# Autodesk Inventor assembly: CE-9.1.1
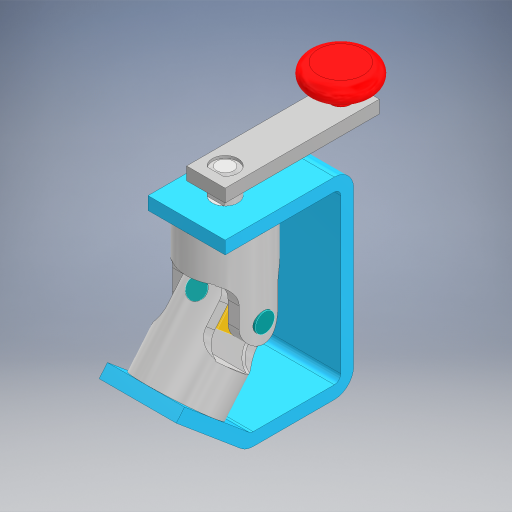
[picture p0: Inventor's stored thumbnail of the model, 512x512]
Saved by Autodesk Inventor 2024 (Build 280153000, 153)
## iProperties
Created: 2024-03-14
Part Number: CE-9.1.1
Document SubType Name: Assembly
Designer: Alex
Author: Alex
## Documents named in this file (9)
- C:\Shared\alex-bartella-schoolwork\4z03\Week 9\CE-9.1.1.iam
- C:\Shared\alex-bartella-schoolwork\4z03\Week 9\STEP\CE-9.1.1 STEP Files\bracket\bracket.ipt
- C:\Shared\alex-bartella-schoolwork\4z03\Week 9\STEP\CE-9.1.1 STEP Files\Yoke_F\Yoke_F.ipt
- C:\Shared\alex-bartella-schoolwork\4z03\Week 9\STEP\CE-9.1.1 STEP Files\Yoke_M\Yoke_M.ipt
- C:\Shared\alex-bartella-schoolwork\4z03\Week 9\STEP\CE-9.1.1 STEP Files\spider\spider.ipt
- C:\Shared\alex-bartella-schoolwork\4z03\Week 9\STEP\CE-9.1.1 STEP Files\arm\arm.ipt
- C:\Shared\alex-bartella-schoolwork\4z03\Week 9\STEP\CE-9.1.1 STEP Files\knob\knob.ipt
- C:\Shared\alex-bartella-schoolwork\4z03\Week 9\STEP\CE-9.1.1 STEP Files\pin_long\pin_long.ipt
- C:\Shared\alex-bartella-schoolwork\4z03\Week 9\STEP\CE-9.1.1 STEP Files\pin_short\pin_short.ipt
## Components (9 placed, 8 different names)
1. bracket:1 — Flush:1, Flush:2, Flush:3, Mate:1, Mate:2, Angle:1, Angle:4
2. Yoke_F:1 — Angle:1, Mate:4, Mate:6, Mate:13
3. Yoke_M:1 — Mate:1, Mate:2, Mate:3, Mate:5, Angle:3, Mate:8, Mate:11, Mate:12, Flush:7
4. spider:1 — Mate:3, Mate:4, Mate:5, Mate:6, Flush:4, Flush:5, Flush:6
5. arm:1 — Angle:3, Mate:8, Mate:9, Mate:10, Flush:7, Angle:4
6. knob:1 — Mate:9, Mate:10
7. pin_long:1 — Mate:13, Flush:6
8. pin_short:1 — Mate:12, Flush:4
9. pin_short:2 — Mate:11, Flush:5
## Relationships (22: Mate 12, Flush 7, Angle 3)
- Flush:1: bracket:1
- Flush:2: bracket:1
- Flush:3: bracket:1
- Mate:1: bracket:1 ↔ Yoke_M:1
- Mate:2: bracket:1 ↔ Yoke_M:1
- Angle:1 (180 deg): bracket:1 ↔ Yoke_F:1
- Mate:3: Yoke_M:1 ↔ spider:1
- Mate:4: Yoke_F:1 ↔ spider:1
- Mate:5 (0.5 mm): Yoke_M:1 ↔ spider:1
- Mate:6 (0.5 mm): Yoke_F:1 ↔ spider:1
- Angle:3 (180 deg): Yoke_M:1 ↔ arm:1
- Mate:8: Yoke_M:1 ↔ arm:1
- Mate:9: arm:1 ↔ knob:1
- Mate:10: arm:1 ↔ knob:1
- Mate:11: Yoke_M:1 ↔ pin_short:2
- Mate:12: Yoke_M:1 ↔ pin_short:1
- Flush:4 (-10 mm): spider:1 ↔ pin_short:1
- Flush:5 (-10 mm): spider:1 ↔ pin_short:2
- Mate:13: Yoke_F:1 ↔ pin_long:1
- Flush:6 (10 mm): spider:1 ↔ pin_long:1
- Flush:7: Yoke_M:1 ↔ arm:1
- Angle:4 (0 deg): bracket:1 ↔ arm:1
